# Autodesk Inventor assembly: ASM X-Axis
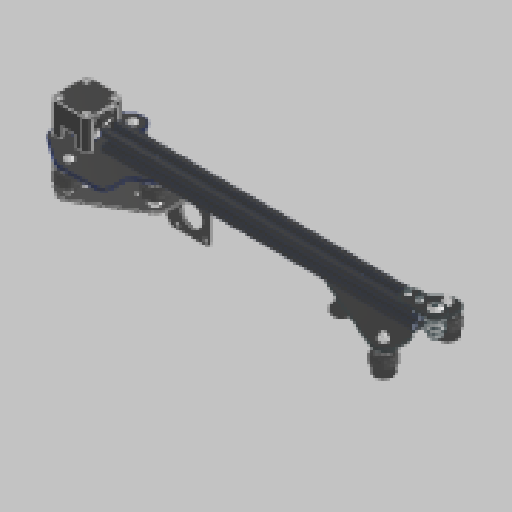
[picture p0: Inventor's stored thumbnail of the model, 512x512]
Saved by Autodesk Inventor 2025.4 (Build 294407000, 407)
## iProperties
Created: 2022-04-13
Part Number: ASM X-Axis
Document SubType Name: Assembly
Designer: javie
Author: javie
Revision Number: ANY
## Documents named in this file (27)
- C:\Users\Inema\OneDrive - INEMA S.A\Escritorio\Modelo Ender 3\ASM X-Axis.iam
- C:\Users\Inema\OneDrive - INEMA S.A\Escritorio\Modelo Ender 3\2020 profile.ipt
- C:\Users\Inema\OneDrive - INEMA S.A\Escritorio\Modelo Ender 3\Z Stent.ipt
- C:\Users\Inema\OneDrive - INEMA S.A\Escritorio\Modelo Ender 3\X motor bracket.ipt
- C:\Users\Inema\OneDrive - INEMA S.A\Escritorio\Modelo Ender 3\42-34 motor.ipt
- C:\Users\Inema\OneDrive - INEMA S.A\Escritorio\Modelo Ender 3\z nut.ipt
- C:\Users\Inema\OneDrive - INEMA S.A\Escritorio\Modelo Ender 3\E motor bracket.ipt
- C:\Users\Inema\OneDrive - INEMA S.A\Escritorio\Modelo Ender 3\X limit switch bracket.ipt
- C:\Users\Inema\OneDrive - INEMA S.A\Escritorio\Modelo Ender 3\X belt.ipt
- C:\Users\Inema\OneDrive - INEMA S.A\Escritorio\Modelo Ender 3\limit switch.ipt
- C:\Users\Inema\OneDrive - INEMA S.A\Escritorio\Modelo Ender 3\2GT-pulley.ipt
- C:\Users\Inema\OneDrive - INEMA S.A\Escritorio\Modelo Ender 3\Copper cover.ipt
- C:\Users\Inema\OneDrive - INEMA S.A\Escritorio\Modelo Ender 3\M4 Split Washer.ipt
- C:\Users\Inema\OneDrive - INEMA S.A\Escritorio\Modelo Ender 3\M3 Split Washer.ipt
- C:\Users\Inema\OneDrive - INEMA S.A\Escritorio\Modelo Ender 3\M4X16 Pan Head Screw.ipt
- C:\Users\Inema\OneDrive - INEMA S.A\Escritorio\Modelo Ender 3\M3X40-P.ipt
- C:\Users\Inema\OneDrive - INEMA S.A\Escritorio\Modelo Ender 3\M3X10 Pan Head Screw.ipt
- C:\Users\Inema\OneDrive - INEMA S.A\Escritorio\Modelo Ender 3\M3X6Pan Head Screw.ipt
- C:\Users\Inema\OneDrive - INEMA S.A\Escritorio\Modelo Ender 3\ASM Eccentrical Roller Z-Axis Left.iam
- C:\Users\Inema\OneDrive - INEMA S.A\Escritorio\Modelo Ender 3\ASM Roller Z-Axis Left.iam
- C:\Users\Inema\OneDrive - INEMA S.A\Escritorio\Modelo Ender 3\ASM X-Belt Tensioner.iam
- C:\Users\Inema\OneDrive - INEMA S.A\Escritorio\Modelo Ender 3\ASM Eccentrical Roller Z-Axis Right.iam
- C:\Users\Inema\OneDrive - INEMA S.A\Escritorio\Modelo Ender 3\ASM Roller Z-Axis Right.iam
- C:\Users\Inema\OneDrive - INEMA S.A\Escritorio\Modelo Ender 3\Ender_3_Fan_Duct_-_V59\Ender_3_Fan_Duct_-_V59\Ender 3 Fan Duct.iam
- C:\Users\Inema\OneDrive - INEMA S.A\Escritorio\Modelo Ender 3\M5 Self-locking nut.ipt
- C:\Users\Inema\OneDrive - INEMA S.A\Escritorio\Modelo Ender 3\Spacer1.ipt
- C:\Users\Inema\OneDrive - INEMA S.A\Escritorio\Modelo Ender 3\Spacer2.ipt
## Components (42 placed, 41 different names)
1. 2020 profile_129
2. Z Stent_130 — Insertar:2
3. X motor bracket_131
4. 42-34 motor_132
5. z nut_133
6. E motor bracket_134
7. X limit switch bracket_135
8. X belt_136
9. limit switch_137
10. 2GT-pulley_138
11. Copper cover_139
12. Copper cover_140
13. M4 Split Washer_141
14. M4 Split Washer_142
15. M3 Split Washer_143
16. M4X16 Pan Head Screw_144
17. M3X40-P_145
18. M4X16 Pan Head Screw_146
19. M3X40-P_147
20. M3X40-P_148
21. M3X40-P_149
22. M4X16 Pan Head Screw_150
23. M4 Split Washer_151
24. M4X16 Pan Head Screw_152
25. M4 Split Washer_153
26. M3X10 Pan Head Screw_154
27. M3 Split Washer_155
28. M3X10 Pan Head Screw_156
29. M3X6Pan Head Screw_157
30. M3X6Pan Head Screw_158
31. ASM Eccentrical Roller Z-Axis Left_159 [sub-assembly]
32. ASM Roller Z-Axis Left_160 [sub-assembly]
33. ASM Roller Z-Axis Left_161 [sub-assembly]
34. ASM X-Belt Tensioner_163 [sub-assembly]
35. ASM Eccentrical Roller Z-Axis Right_164 [sub-assembly] — Insertar:1
36. ASM Roller Z-Axis Right_165 [sub-assembly] — Insertar:3
37. ASM Roller Z-Axis Right_166 [sub-assembly] — Insertar:4
38. Ender 3 Fan Duct:1 [sub-assembly]
39. M5 Self-locking nut_225 — Insertar:1
40. Spacer1:1 — Insertar:2
41. Spacer2:1 — Insertar:3
42. Spacer2:2 — Insertar:4
## Relationships (4: Insert 4)
- Insertar:1: ASM Eccentrical Roller Z-Axis Right_164 ↔ M5 Self-locking nut_225
- Insertar:2: Z Stent_130 ↔ Spacer1:1
- Insertar:3: ASM Roller Z-Axis Right_165 ↔ Spacer2:1
- Insertar:4: ASM Roller Z-Axis Right_166 ↔ Spacer2:2
